# Autodesk Inventor assembly: hex_nut_retainer_w_lock_nut
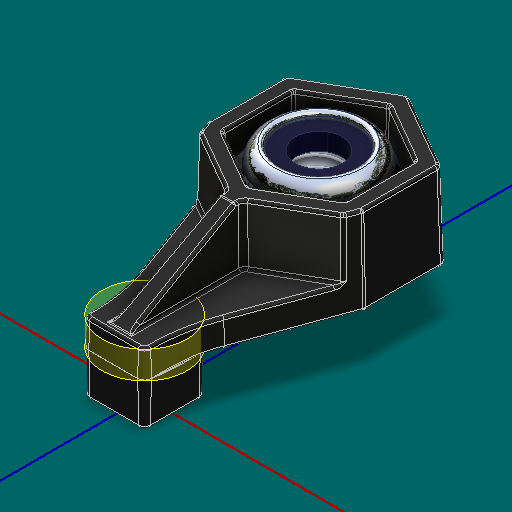
[picture p0: Inventor's stored thumbnail of the model, 512x512]
Saved by Autodesk Inventor 2025 (Build 290162000, 162)
## iProperties
Created: 2024-08-18
Part Number: hex_nut_retainer_w_lock_nut
Document SubType Name: Assembly
Designer: averey
Author: averey
## Documents named in this file (3)
- C:\Users\avere\vex_robotics_high_stakes\hardware\cad\_quick_assemblies\hex_nut_retainer_w_lock_nut.iam
- C:\Users\avere\vex_robotics_high_stakes\hardware\cad\VEX-CAD-Inventor\Structure\1-Post Hex Nut Retainer.ipt
- C:\Users\avere\vex_robotics_high_stakes\hardware\cad\VEX-CAD-Inventor\Structure\Hardware\Nut Thin Nylock.ipt
## Components (2 placed, 2 different names)
1. 1-Post Hex Nut Retainer:1 — Mate:1, Insert:1
2. Nut Thin Nylock:1 — Insert:1
## Relationships (2: Mate 1, Insert 1)
- Mate:1: 1-Post Hex Nut Retainer:1
- Insert:1: 1-Post Hex Nut Retainer:1 ↔ Nut Thin Nylock:1
